# Autodesk Inventor assembly: Body
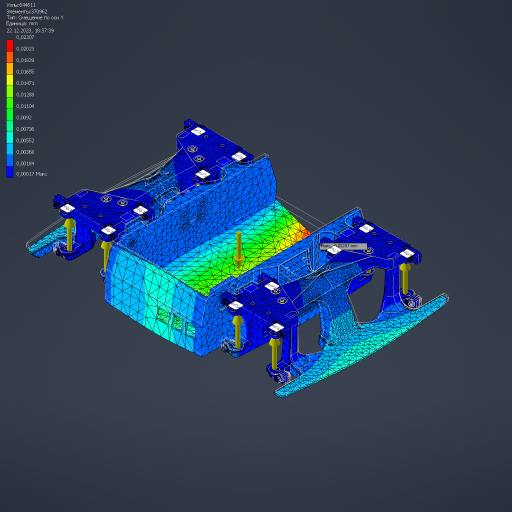
[picture p0: Inventor's stored thumbnail of the model, 512x512]
Saved by Autodesk Inventor 2023 (Build 270158000, 158)
## iProperties
Created: 2023-07-04
Part Number: Body
Document SubType Name: Assembly
Designer: khrip
Mass: 1155.31 g
Surface Area: 2834.72 cm^2
Volume: 832.799 cm^3
Density: 1.38726 g/cm^3
Author: khrip
## Documents named in this file (18)
- C:\GitHub\Botik\Body.iam
- C:\GitHub\Botik\BodyPlate.ipt
- C:\GitHub\Botik\BodyCupDiassembled.ipt
- C:\GitHub\Botik\BodyCupDiassembledMirrored.ipt
- C:\GitHub\Botik\Bumper.ipt
- C:\Users\khrip\OneDrive\Документы\Inventor\Content Center Files\R2023\ru-RU\GOST 11371-78  A\Шайба 3 ГОСТ 11371-78.ipt
- C:\Users\khrip\OneDrive\Документы\Inventor\Content Center Files\R2023\ru-RU\DIN 934\DIN 934 - M3 x 0,5.ipt
- C:\Users\khrip\OneDrive\Документы\Inventor\Content Center Files\R2023\ru-RU\DIN 912\DIN 912 - M3 x 0,5 x 10 x 8,75.ipt
- C:\GitHub\Botik\CrossBar.ipt
- C:\Users\khrip\OneDrive\Документы\Inventor\Content Center Files\R2023\ru-RU\GOST 17475-80 (2)\Винт 2.M4-6gx14 ГОСТ 17475-80.ipt
- C:\Users\khrip\OneDrive\Документы\Inventor\Content Center Files\R2023\ru-RU\GOST 11371-78  A\Шайба 4 ГОСТ 11371-78.ipt
- C:\Users\khrip\OneDrive\Документы\Inventor\Content Center Files\R2023\ru-RU\DIN 934\DIN 934 - M4 x 0,7.ipt
- C:\GitHub\Botik\Body\AIP\FEA\ek0i76urk.fins
- C:\GitHub\Botik\Body\AIP\FEA\ek0i76urk.fsat
- C:\GitHub\Botik\Body\AIP\FEA\ek0i76urk.ftes
- C:\GitHub\Botik\Body\AIP\FEA\ek0i76urk.fwiz
- C:\GitHub\Botik\Body\AIP\FEA\ek0i76v5s.fmsh
- C:\GitHub\Botik\Body\AIP\FEA\ek0i76v5t.fres
## Components (145 placed, 11 different names)
1. BodyPlate:1 — Совмещение:40, Заподлицо:14, Совмещение:41, Совмещение:42, Совмещение:43, Заподлицо:15, Совмещение:44, Заподлицо:16, Совмещение:45, Заподлицо:17, Совмещение:47, Совмещение:48, Вставка:4, Вставка:5, Вставка:9, Вставка:10, Вставка:12, Вставка:13, Вставка:15, Вставка:16, Вставка:17, Вставка:18, Вставка:19, Вставка:20, Вставка:24, Вставка:25, Вставка:27, Вставка:28
2. BodyCupDiassembled:1 — Совмещение:40, Заподлицо:14, Совмещение:41, Совмещение:51, Совмещение:52, Заподлицо:19, Вставка:30, Вставка:31, Вставка:32, Вставка:33, Вставка:34, Вставка:35, Совмещение:159, Совмещение:162, Совмещение:163, Совмещение:171, Совмещение:173
3. BodyCupDiassembled:2 — Совмещение:42, Совмещение:43, Заподлицо:15, Совмещение:49, Совмещение:50, Заподлицо:18, Совмещение:53, Совмещение:54, Совмещение:55, Совмещение:56, Вставка:21, Вставка:22, Вставка:23, Вставка:26, Совмещение:166, Совмещение:167, Совмещение:179, Совмещение:181
4. BodyCupDiassembledMirroredMirrored:1 — Заподлицо:17, Совмещение:47, Совмещение:48, Вставка:2, Вставка:3, Вставка:7, Вставка:8, Вставка:11, Вставка:14, Совмещение:168, Совмещение:169, Совмещение:183, Совмещение:185
5. BodyCupDiassembledMirroredMirrored:2 — Совмещение:44, Заподлицо:16, Совмещение:45, Вставка:39, Вставка:40, Вставка:42, Вставка:43, Вставка:44, Вставка:45, Совмещение:160, Совмещение:164, Совмещение:165, Совмещение:175, Совмещение:177
6. Bumper:1 — Совмещение:49, Совмещение:50, Заподлицо:18, Вставка:1, Вставка:6, Совмещение:57, Совмещение:58, Вставка:29, Совмещение:157, Совмещение:158
7. Bumper:2 — Совмещение:51, Совмещение:52, Заподлицо:19, Вставка:36, Вставка:37, Вставка:38, Вставка:41, Совмещение:161
8. CrossBar:1 — Вставка:54, Вставка:55, Вставка:56, Вставка:57, Вставка:58, Вставка:59, Вставка:60, Вставка:61, Совмещение:157, Совмещение:158
9. CrossBar:2 — Вставка:46, Вставка:47, Вставка:48, Вставка:49, Вставка:50, Вставка:51, Вставка:52, Вставка:53, Совмещение:159, Совмещение:160, Совмещение:161
10. DIN 934 - заменено на DIN EN 24032/28673/28674 M3:25 — Вставка:46
11. DIN 934 - заменено на DIN EN 24032/28673/28674 M3:26 — Вставка:47
12. DIN 934 - заменено на DIN EN 24032/28673/28674 M3:27 — Вставка:48
13. DIN 934 - заменено на DIN EN 24032/28673/28674 M3:28 — Вставка:49
14. DIN 934 - заменено на DIN EN 24032/28673/28674 M3:29 — Вставка:50
15. DIN 934 - заменено на DIN EN 24032/28673/28674 M3:30 — Вставка:51
16. DIN 934 - заменено на DIN EN 24032/28673/28674 M3:31 — Вставка:52
17. DIN 934 - заменено на DIN EN 24032/28673/28674 M3:32 — Вставка:53
18. DIN 934 - заменено на DIN EN 24032/28673/28674 M3:33 — Вставка:54
19. DIN 934 - заменено на DIN EN 24032/28673/28674 M3:34 — Вставка:55
20. DIN 934 - заменено на DIN EN 24032/28673/28674 M3:35 — Вставка:56
21. DIN 934 - заменено на DIN EN 24032/28673/28674 M3:36 — Вставка:57
22. DIN 934 - заменено на DIN EN 24032/28673/28674 M3:37 — Вставка:58
23. DIN 934 - заменено на DIN EN 24032/28673/28674 M3:38 — Вставка:59
24. DIN 934 - заменено на DIN EN 24032/28673/28674 M3:39 — Вставка:60
25. DIN 934 - заменено на DIN EN 24032/28673/28674 M3:40 — Вставка:61
26. Винт 2 ГОСТ 17475-80 M4 x 14:1 — Совмещение:162, Совмещение:170, Совмещение:196
27. Винт 2 ГОСТ 17475-80 M4 x 14:2 — Совмещение:163, Совмещение:172, Совмещение:194
28. Винт 2 ГОСТ 17475-80 M4 x 14:3 — Совмещение:164, Совмещение:176, Совмещение:200
29. Винт 2 ГОСТ 17475-80 M4 x 14:4 — Совмещение:165, Совмещение:174, Совмещение:198
30. Винт 2 ГОСТ 17475-80 M4 x 14:5 — Совмещение:166, Совмещение:178, Совмещение:192
31. Винт 2 ГОСТ 17475-80 M4 x 14:6 — Совмещение:167, Совмещение:180, Совмещение:190
32. Винт 2 ГОСТ 17475-80 M4 x 14:7 — Совмещение:168, Совмещение:182, Совмещение:186
33. Винт 2 ГОСТ 17475-80 M4 x 14:8 — Совмещение:169, Совмещение:184, Совмещение:188
34. Шайба  ГОСТ 11371-78 4,3:1 — Совмещение:170, Совмещение:171, Совмещение:197
35. Шайба  ГОСТ 11371-78 4,3:2 — Совмещение:172, Совмещение:173, Совмещение:195
36. Шайба  ГОСТ 11371-78 4,3:3 — Совмещение:174, Совмещение:175, Совмещение:199
37. Шайба  ГОСТ 11371-78 4,3:4 — Совмещение:176, Совмещение:177, Совмещение:201
38. Шайба  ГОСТ 11371-78 4,3:5 — Совмещение:178, Совмещение:179, Совмещение:193
39. Шайба  ГОСТ 11371-78 4,3:6 — Совмещение:180, Совмещение:181, Совмещение:191
40. Шайба  ГОСТ 11371-78 4,3:7 — Совмещение:182, Совмещение:183, Совмещение:187
41. Шайба  ГОСТ 11371-78 4,3:8 — Совмещение:184, Совмещение:185, Совмещение:189
42. DIN 934 - заменено на DIN EN 24032/28673/28674 M4:1 — Совмещение:186, Совмещение:187
43. DIN 934 - заменено на DIN EN 24032/28673/28674 M4:2 — Совмещение:188, Совмещение:189
44. DIN 934 - заменено на DIN EN 24032/28673/28674 M4:3 — Совмещение:190, Совмещение:191
45. DIN 934 - заменено на DIN EN 24032/28673/28674 M4:4 — Совмещение:192, Совмещение:193
46. DIN 934 - заменено на DIN EN 24032/28673/28674 M4:5 — Совмещение:194, Совмещение:195
47. DIN 934 - заменено на DIN EN 24032/28673/28674 M4:6 — Совмещение:196, Совмещение:197
48. DIN 934 - заменено на DIN EN 24032/28673/28674 M4:7 — Совмещение:198, Совмещение:199
49. DIN 934 - заменено на DIN EN 24032/28673/28674 M4:8 — Совмещение:200, Совмещение:201
50. Шайба  ГОСТ 11371-78 3,2:11 — Вставка:11, Совмещение:79, Совмещение:80
51. Шайба  ГОСТ 11371-78 3,2:12 — Вставка:12, Совмещение:81, Совмещение:82
52. Шайба  ГОСТ 11371-78 3,2:13 — Вставка:13, Совмещение:69, Совмещение:70
53. Шайба  ГОСТ 11371-78 3,2:14 — Вставка:14, Совмещение:124
54. Шайба  ГОСТ 11371-78 3,2:15 — Вставка:15, Совмещение:126
55. Шайба  ГОСТ 11371-78 3,2:16 — Вставка:16, Совмещение:118
56. Шайба  ГОСТ 11371-78 3,2:17 — Совмещение:53, Совмещение:54, Совмещение:71, Совмещение:72
57. Шайба  ГОСТ 11371-78 3,2:18 — Совмещение:55, Совмещение:56, Совмещение:73, Совмещение:74
58. Шайба  ГОСТ 11371-78 3,2:19 — Вставка:17, Совмещение:77, Совмещение:78
59. Шайба  ГОСТ 11371-78 3,2:20 — Вставка:18, Совмещение:63, Совмещение:64
60. Шайба  ГОСТ 11371-78 3,2:21 — Вставка:19, Совмещение:128
61. Шайба  ГОСТ 11371-78 3,2:22 — Вставка:20, Совмещение:112
62. Шайба  ГОСТ 11371-78 3,2:23 — Вставка:21, Совмещение:130
63. Шайба  ГОСТ 11371-78 3,2:24 — Вставка:22, Совмещение:96
64. Шайба  ГОСТ 11371-78 3,2:25 — Вставка:23, Совмещение:83, Совмещение:84
65. Шайба  ГОСТ 11371-78 3,2:26 — Вставка:24, Совмещение:85, Совмещение:86
66. Шайба  ГОСТ 11371-78 3,2:27 — Вставка:25, Совмещение:99, Совмещение:100
67. Шайба  ГОСТ 11371-78 3,2:28 — Вставка:26, Совмещение:142
68. Шайба  ГОСТ 11371-78 3,2:29 — Вставка:27, Совмещение:140
69. Шайба  ГОСТ 11371-78 3,2:30 — Вставка:28, Совмещение:152
70. Шайба  ГОСТ 11371-78 3,2:31 — Совмещение:57, Совмещение:58, Совмещение:75, Совмещение:76
71. Шайба  ГОСТ 11371-78 3,2:32 — Вставка:29, Совмещение:110
72. Шайба  ГОСТ 11371-78 3,2:33 — Вставка:30, Совмещение:101, Совмещение:102
73. Шайба  ГОСТ 11371-78 3,2:34 — Вставка:31, Совмещение:105, Совмещение:106
74. Шайба  ГОСТ 11371-78 3,2:35 — Вставка:32, Совмещение:136
75. Шайба  ГОСТ 11371-78 3,2:36 — Вставка:33, Совмещение:134
76. Шайба  ГОСТ 11371-78 3,2:37 — Вставка:34, Совмещение:67, Совмещение:68
77. Шайба  ГОСТ 11371-78 3,2:38 — Вставка:35, Совмещение:116
78. Шайба  ГОСТ 11371-78 3,2:39 — Вставка:36, Совмещение:132
79. Шайба  ГОСТ 11371-78 3,2:40 — Вставка:37, Совмещение:107, Совмещение:108
80. Шайба  ГОСТ 11371-78 3,2:41 — Вставка:38, Совмещение:65, Совмещение:66
81. Шайба  ГОСТ 11371-78 3,2:42 — Вставка:39, Совмещение:61, Совмещение:62
82. Шайба  ГОСТ 11371-78 3,2:43 — Вставка:40, Совмещение:59, Совмещение:60
83. Шайба  ГОСТ 11371-78 3,2:44 — Вставка:41, Совмещение:122
84. Шайба  ГОСТ 11371-78 3,2:45 — Вставка:42, Совмещение:120
85. Шайба  ГОСТ 11371-78 3,2:46 — Вставка:43, Совмещение:114
86. Шайба  ГОСТ 11371-78 3,2:47 — Вставка:44, Совмещение:138
87. Шайба  ГОСТ 11371-78 3,2:48 — Вставка:45, Совмещение:97, Совмещение:98
88. Шайба  ГОСТ 11371-78 3,2:1 — Вставка:1, Совмещение:89, Совмещение:90
89. Шайба  ГОСТ 11371-78 3,2:2 — Вставка:2, Совмещение:87, Совмещение:88
90. Шайба  ГОСТ 11371-78 3,2:3 — Вставка:3, Совмещение:91, Совмещение:92
91. Шайба  ГОСТ 11371-78 3,2:4 — Вставка:4, Совмещение:93, Совмещение:94
92. Шайба  ГОСТ 11371-78 3,2:5 — Вставка:5, Совмещение:103, Совмещение:104
93. Шайба  ГОСТ 11371-78 3,2:6 — Вставка:6, Совмещение:148
94. Шайба  ГОСТ 11371-78 3,2:7 — Вставка:7, Совмещение:150
95. Шайба  ГОСТ 11371-78 3,2:8 — Вставка:8, Совмещение:144
96. Шайба  ГОСТ 11371-78 3,2:9 — Вставка:9, Совмещение:146
97. Шайба  ГОСТ 11371-78 3,2:10 — Вставка:10, Совмещение:154
98. DIN 912 - заменено на DIN EN ISO 4762 M3 x 10:1 — Совмещение:59, Совмещение:60, Совмещение:113
99. DIN 912 - заменено на DIN EN ISO 4762 M3 x 10:2 — Совмещение:61, Совмещение:62, Совмещение:119
100. DIN 912 - заменено на DIN EN ISO 4762 M3 x 10:3 — Совмещение:63, Совмещение:64, Совмещение:111
101. DIN 912 - заменено на DIN EN ISO 4762 M3 x 10:4 — Совмещение:65, Совмещение:66, Совмещение:121
102. DIN 912 - заменено на DIN EN ISO 4762 M3 x 10:5 — Совмещение:67, Совмещение:68, Совмещение:115
103. DIN 912 - заменено на DIN EN ISO 4762 M3 x 10:6 — Совмещение:69, Совмещение:70, Совмещение:117
104. DIN 912 - заменено на DIN EN ISO 4762 M3 x 10:7 — Совмещение:71, Совмещение:72, Совмещение:129
105. DIN 912 - заменено на DIN EN ISO 4762 M3 x 10:8 — Совмещение:73, Совмещение:74, Совмещение:95
106. DIN 912 - заменено на DIN EN ISO 4762 M3 x 10:9 — Совмещение:75, Совмещение:76, Совмещение:109
107. DIN 912 - заменено на DIN EN ISO 4762 M3 x 10:10 — Совмещение:77, Совмещение:78, Совмещение:127
108. DIN 912 - заменено на DIN EN ISO 4762 M3 x 10:11 — Совмещение:79, Совмещение:80, Совмещение:123
109. DIN 912 - заменено на DIN EN ISO 4762 M3 x 10:12 — Совмещение:81, Совмещение:82, Совмещение:125
110. DIN 912 - заменено на DIN EN ISO 4762 M3 x 10:13 — Совмещение:83, Совмещение:84, Совмещение:141
111. DIN 912 - заменено на DIN EN ISO 4762 M3 x 10:14 — Совмещение:85, Совмещение:86, Совмещение:139
112. DIN 912 - заменено на DIN EN ISO 4762 M3 x 10:15 — Совмещение:87, Совмещение:88, Совмещение:149
113. DIN 912 - заменено на DIN EN ISO 4762 M3 x 10:16 — Совмещение:89, Совмещение:90, Совмещение:147
114. DIN 912 - заменено на DIN EN ISO 4762 M3 x 10:17 — Совмещение:91, Совмещение:92, Совмещение:143
115. DIN 912 - заменено на DIN EN ISO 4762 M3 x 10:18 — Совмещение:93, Совмещение:94, Совмещение:145
116. DIN 912 - заменено на DIN EN ISO 4762 M3 x 10:19 — Совмещение:97, Совмещение:98, Совмещение:137
117. DIN 912 - заменено на DIN EN ISO 4762 M3 x 10:20 — Совмещение:99, Совмещение:100, Совмещение:151
118. DIN 912 - заменено на DIN EN ISO 4762 M3 x 10:21 — Совмещение:101, Совмещение:102, Совмещение:135
119. DIN 912 - заменено на DIN EN ISO 4762 M3 x 10:22 — Совмещение:103, Совмещение:104, Совмещение:153
120. DIN 912 - заменено на DIN EN ISO 4762 M3 x 10:23 — Совмещение:105, Совмещение:106, Совмещение:133
121. DIN 912 - заменено на DIN EN ISO 4762 M3 x 10:24 — Совмещение:107, Совмещение:108, Совмещение:131
122. DIN 934 - заменено на DIN EN 24032/28673/28674 M3:2 — Совмещение:109, Совмещение:110
123. DIN 934 - заменено на DIN EN 24032/28673/28674 M3:3 — Совмещение:111, Совмещение:112
124. DIN 934 - заменено на DIN EN 24032/28673/28674 M3:4 — Совмещение:113, Совмещение:114
125. DIN 934 - заменено на DIN EN 24032/28673/28674 M3:5 — Совмещение:115, Совмещение:116
126. DIN 934 - заменено на DIN EN 24032/28673/28674 M3:6 — Совмещение:117, Совмещение:118
127. DIN 934 - заменено на DIN EN 24032/28673/28674 M3:7 — Совмещение:119, Совмещение:120
128. DIN 934 - заменено на DIN EN 24032/28673/28674 M3:8 — Совмещение:121, Совмещение:122
129. DIN 934 - заменено на DIN EN 24032/28673/28674 M3:9 — Совмещение:123, Совмещение:124
130. DIN 934 - заменено на DIN EN 24032/28673/28674 M3:10 — Совмещение:125, Совмещение:126
131. DIN 934 - заменено на DIN EN 24032/28673/28674 M3:11 — Совмещение:127, Совмещение:128
132. DIN 934 - заменено на DIN EN 24032/28673/28674 M3:12 — Совмещение:129, Совмещение:130
133. DIN 934 - заменено на DIN EN 24032/28673/28674 M3:13 — Совмещение:131, Совмещение:132
134. DIN 934 - заменено на DIN EN 24032/28673/28674 M3:14 — Совмещение:133, Совмещение:134
135. DIN 934 - заменено на DIN EN 24032/28673/28674 M3:15 — Совмещение:135, Совмещение:136
136. DIN 934 - заменено на DIN EN 24032/28673/28674 M3:16 — Совмещение:137, Совмещение:138
137. DIN 934 - заменено на DIN EN 24032/28673/28674 M3:17 — Совмещение:139, Совмещение:140
138. DIN 934 - заменено на DIN EN 24032/28673/28674 M3:18 — Совмещение:141, Совмещение:142
139. DIN 934 - заменено на DIN EN 24032/28673/28674 M3:19 — Совмещение:143, Совмещение:144
140. DIN 934 - заменено на DIN EN 24032/28673/28674 M3:20 — Совмещение:145, Совмещение:146
141. DIN 934 - заменено на DIN EN 24032/28673/28674 M3:21 — Совмещение:147, Совмещение:148
142. DIN 934 - заменено на DIN EN 24032/28673/28674 M3:22 — Совмещение:149, Совмещение:150
143. DIN 934 - заменено на DIN EN 24032/28673/28674 M3:23 — Совмещение:151, Совмещение:152
144. DIN 934 - заменено на DIN EN 24032/28673/28674 M3:24 — Совмещение:153, Совмещение:154
145. DIN 934 - заменено на DIN EN 24032/28673/28674 M3:1 — Совмещение:95, Совмещение:96
## Relationships (226: Mate 159, Insert 61, Flush 6)
- Совмещение:40 [Mate]: BodyPlate:1 ↔ BodyCupDiassembled:1
- Заподлицо:14 [Flush]: BodyPlate:1 ↔ BodyCupDiassembled:1
- Совмещение:41 [Mate]: BodyPlate:1 ↔ BodyCupDiassembled:1
- Совмещение:42 [Mate]: BodyPlate:1 ↔ BodyCupDiassembled:2
- Совмещение:43 [Mate]: BodyPlate:1 ↔ BodyCupDiassembled:2
- Заподлицо:15 [Flush]: BodyPlate:1 ↔ BodyCupDiassembled:2
- Совмещение:44 [Mate]: BodyPlate:1 ↔ BodyCupDiassembledMirroredMirrored:2
- Заподлицо:16 [Flush]: BodyPlate:1 ↔ BodyCupDiassembledMirroredMirrored:2
- Совмещение:45 [Mate]: BodyPlate:1 ↔ BodyCupDiassembledMirroredMirrored:2
- Заподлицо:17 [Flush]: BodyPlate:1 ↔ BodyCupDiassembledMirroredMirrored:1
- Совмещение:47 [Mate]: BodyPlate:1 ↔ BodyCupDiassembledMirroredMirrored:1
- Совмещение:48 [Mate]: BodyPlate:1 ↔ BodyCupDiassembledMirroredMirrored:1
- Совмещение:49 [Mate]: BodyCupDiassembled:2 ↔ Bumper:1
- Совмещение:50 [Mate]: BodyCupDiassembled:2 ↔ Bumper:1
- Заподлицо:18 [Flush]: BodyCupDiassembled:2 ↔ Bumper:1
- Совмещение:51 [Mate]: BodyCupDiassembled:1 ↔ Bumper:2
- Совмещение:52 [Mate]: BodyCupDiassembled:1 ↔ Bumper:2
- Заподлицо:19 [Flush]: BodyCupDiassembled:1 ↔ Bumper:2
- Вставка:1 [Insert]: Bumper:1 ↔ Шайба  ГОСТ 11371-78 3,2:1
- Вставка:2 [Insert]: BodyCupDiassembledMirroredMirrored:1 ↔ Шайба  ГОСТ 11371-78 3,2:2
- Вставка:3 [Insert]: BodyCupDiassembledMirroredMirrored:1 ↔ Шайба  ГОСТ 11371-78 3,2:3
- Вставка:4 [Insert]: BodyPlate:1 ↔ Шайба  ГОСТ 11371-78 3,2:4
- Вставка:5 [Insert]: BodyPlate:1 ↔ Шайба  ГОСТ 11371-78 3,2:5
- Вставка:6 [Insert]: Bumper:1 ↔ Шайба  ГОСТ 11371-78 3,2:6
- Вставка:7 [Insert]: BodyCupDiassembledMirroredMirrored:1 ↔ Шайба  ГОСТ 11371-78 3,2:7
- Вставка:8 [Insert]: BodyCupDiassembledMirroredMirrored:1 ↔ Шайба  ГОСТ 11371-78 3,2:8
- Вставка:9 [Insert]: BodyPlate:1 ↔ Шайба  ГОСТ 11371-78 3,2:9
- Вставка:10 [Insert]: BodyPlate:1 ↔ Шайба  ГОСТ 11371-78 3,2:10
- Вставка:11 [Insert]: BodyCupDiassembledMirroredMirrored:1 ↔ Шайба  ГОСТ 11371-78 3,2:11
- Вставка:12 [Insert]: BodyPlate:1 ↔ Шайба  ГОСТ 11371-78 3,2:12
- Вставка:13 [Insert]: BodyPlate:1 ↔ Шайба  ГОСТ 11371-78 3,2:13
- Вставка:14 [Insert]: BodyCupDiassembledMirroredMirrored:1 ↔ Шайба  ГОСТ 11371-78 3,2:14
- Вставка:15 [Insert]: BodyPlate:1 ↔ Шайба  ГОСТ 11371-78 3,2:15
- Вставка:16 [Insert]: BodyPlate:1 ↔ Шайба  ГОСТ 11371-78 3,2:16
- Совмещение:53 [Mate]: BodyCupDiassembled:2 ↔ Шайба  ГОСТ 11371-78 3,2:17
- Совмещение:54 [Mate]: BodyCupDiassembled:2 ↔ Шайба  ГОСТ 11371-78 3,2:17
- Совмещение:55 [Mate]: BodyCupDiassembled:2 ↔ Шайба  ГОСТ 11371-78 3,2:18
- Совмещение:56 [Mate]: BodyCupDiassembled:2 ↔ Шайба  ГОСТ 11371-78 3,2:18
- Вставка:17 [Insert]: BodyPlate:1 ↔ Шайба  ГОСТ 11371-78 3,2:19
- Вставка:18 [Insert]: BodyPlate:1 ↔ Шайба  ГОСТ 11371-78 3,2:20
- Вставка:19 [Insert]: BodyPlate:1 ↔ Шайба  ГОСТ 11371-78 3,2:21
- Вставка:20 [Insert]: BodyPlate:1 ↔ Шайба  ГОСТ 11371-78 3,2:22
- Вставка:21 [Insert]: BodyCupDiassembled:2 ↔ Шайба  ГОСТ 11371-78 3,2:23
- Вставка:22 [Insert]: BodyCupDiassembled:2 ↔ Шайба  ГОСТ 11371-78 3,2:24
- Вставка:23 [Insert]: BodyCupDiassembled:2 ↔ Шайба  ГОСТ 11371-78 3,2:25
- Вставка:24 [Insert]: BodyPlate:1 ↔ Шайба  ГОСТ 11371-78 3,2:26
- Вставка:25 [Insert]: BodyPlate:1 ↔ Шайба  ГОСТ 11371-78 3,2:27
- Вставка:26 [Insert]: BodyCupDiassembled:2 ↔ Шайба  ГОСТ 11371-78 3,2:28
- Вставка:27 [Insert]: BodyPlate:1 ↔ Шайба  ГОСТ 11371-78 3,2:29
- Вставка:28 [Insert]: BodyPlate:1 ↔ Шайба  ГОСТ 11371-78 3,2:30
- Совмещение:57 [Mate]: Bumper:1 ↔ Шайба  ГОСТ 11371-78 3,2:31
- Совмещение:58 [Mate]: Bumper:1 ↔ Шайба  ГОСТ 11371-78 3,2:31
- Вставка:29 [Insert]: Bumper:1 ↔ Шайба  ГОСТ 11371-78 3,2:32
- Вставка:30 [Insert]: BodyCupDiassembled:1 ↔ Шайба  ГОСТ 11371-78 3,2:33
- Вставка:31 [Insert]: BodyCupDiassembled:1 ↔ Шайба  ГОСТ 11371-78 3,2:34
- Вставка:32 [Insert]: BodyCupDiassembled:1 ↔ Шайба  ГОСТ 11371-78 3,2:35
- Вставка:33 [Insert]: BodyCupDiassembled:1 ↔ Шайба  ГОСТ 11371-78 3,2:36
- Вставка:34 [Insert]: BodyCupDiassembled:1 ↔ Шайба  ГОСТ 11371-78 3,2:37
- Вставка:35 [Insert]: BodyCupDiassembled:1 ↔ Шайба  ГОСТ 11371-78 3,2:38
- Вставка:36 [Insert]: Bumper:2 ↔ Шайба  ГОСТ 11371-78 3,2:39
- Вставка:37 [Insert]: Bumper:2 ↔ Шайба  ГОСТ 11371-78 3,2:40
- Вставка:38 [Insert]: Bumper:2 ↔ Шайба  ГОСТ 11371-78 3,2:41
- Вставка:39 [Insert]: BodyCupDiassembledMirroredMirrored:2 ↔ Шайба  ГОСТ 11371-78 3,2:42
- Вставка:40 [Insert]: BodyCupDiassembledMirroredMirrored:2 ↔ Шайба  ГОСТ 11371-78 3,2:43
- Вставка:41 [Insert]: Bumper:2 ↔ Шайба  ГОСТ 11371-78 3,2:44
- Вставка:42 [Insert]: BodyCupDiassembledMirroredMirrored:2 ↔ Шайба  ГОСТ 11371-78 3,2:45
- Вставка:43 [Insert]: BodyCupDiassembledMirroredMirrored:2 ↔ Шайба  ГОСТ 11371-78 3,2:46
- Вставка:44 [Insert]: BodyCupDiassembledMirroredMirrored:2 ↔ Шайба  ГОСТ 11371-78 3,2:47
- Вставка:45 [Insert]: BodyCupDiassembledMirroredMirrored:2 ↔ Шайба  ГОСТ 11371-78 3,2:48
- Совмещение:59 [Mate]: Шайба  ГОСТ 11371-78 3,2:43 ↔ DIN 912 - заменено на DIN EN ISO 4762 M3 x 10:1
- Совмещение:60 [Mate]: Шайба  ГОСТ 11371-78 3,2:43 ↔ DIN 912 - заменено на DIN EN ISO 4762 M3 x 10:1
- Совмещение:61 [Mate]: Шайба  ГОСТ 11371-78 3,2:42 ↔ DIN 912 - заменено на DIN EN ISO 4762 M3 x 10:2
- Совмещение:62 [Mate]: Шайба  ГОСТ 11371-78 3,2:42 ↔ DIN 912 - заменено на DIN EN ISO 4762 M3 x 10:2
- Совмещение:63 [Mate]: Шайба  ГОСТ 11371-78 3,2:20 ↔ DIN 912 - заменено на DIN EN ISO 4762 M3 x 10:3
- Совмещение:64 [Mate]: Шайба  ГОСТ 11371-78 3,2:20 ↔ DIN 912 - заменено на DIN EN ISO 4762 M3 x 10:3
- Совмещение:65 [Mate]: Шайба  ГОСТ 11371-78 3,2:41 ↔ DIN 912 - заменено на DIN EN ISO 4762 M3 x 10:4
- Совмещение:66 [Mate]: Шайба  ГОСТ 11371-78 3,2:41 ↔ DIN 912 - заменено на DIN EN ISO 4762 M3 x 10:4
- Совмещение:67 [Mate]: Шайба  ГОСТ 11371-78 3,2:37 ↔ DIN 912 - заменено на DIN EN ISO 4762 M3 x 10:5
- Совмещение:68 [Mate]: Шайба  ГОСТ 11371-78 3,2:37 ↔ DIN 912 - заменено на DIN EN ISO 4762 M3 x 10:5
- Совмещение:69 [Mate]: Шайба  ГОСТ 11371-78 3,2:13 ↔ DIN 912 - заменено на DIN EN ISO 4762 M3 x 10:6
- Совмещение:70 [Mate]: Шайба  ГОСТ 11371-78 3,2:13 ↔ DIN 912 - заменено на DIN EN ISO 4762 M3 x 10:6
- Совмещение:71 [Mate]: Шайба  ГОСТ 11371-78 3,2:17 ↔ DIN 912 - заменено на DIN EN ISO 4762 M3 x 10:7
- Совмещение:72 [Mate]: Шайба  ГОСТ 11371-78 3,2:17 ↔ DIN 912 - заменено на DIN EN ISO 4762 M3 x 10:7
- Совмещение:73 [Mate]: Шайба  ГОСТ 11371-78 3,2:18 ↔ DIN 912 - заменено на DIN EN ISO 4762 M3 x 10:8
- Совмещение:74 [Mate]: Шайба  ГОСТ 11371-78 3,2:18 ↔ DIN 912 - заменено на DIN EN ISO 4762 M3 x 10:8
- Совмещение:75 [Mate]: Шайба  ГОСТ 11371-78 3,2:31 ↔ DIN 912 - заменено на DIN EN ISO 4762 M3 x 10:9
- Совмещение:76 [Mate]: Шайба  ГОСТ 11371-78 3,2:31 ↔ DIN 912 - заменено на DIN EN ISO 4762 M3 x 10:9
- Совмещение:77 [Mate]: Шайба  ГОСТ 11371-78 3,2:19 ↔ DIN 912 - заменено на DIN EN ISO 4762 M3 x 10:10
- Совмещение:78 [Mate]: Шайба  ГОСТ 11371-78 3,2:19 ↔ DIN 912 - заменено на DIN EN ISO 4762 M3 x 10:10
- Совмещение:79 [Mate]: Шайба  ГОСТ 11371-78 3,2:11 ↔ DIN 912 - заменено на DIN EN ISO 4762 M3 x 10:11
- Совмещение:80 [Mate]: Шайба  ГОСТ 11371-78 3,2:11 ↔ DIN 912 - заменено на DIN EN ISO 4762 M3 x 10:11
- Совмещение:81 [Mate]: Шайба  ГОСТ 11371-78 3,2:12 ↔ DIN 912 - заменено на DIN EN ISO 4762 M3 x 10:12
- Совмещение:82 [Mate]: Шайба  ГОСТ 11371-78 3,2:12 ↔ DIN 912 - заменено на DIN EN ISO 4762 M3 x 10:12
- Совмещение:83 [Mate]: Шайба  ГОСТ 11371-78 3,2:25 ↔ DIN 912 - заменено на DIN EN ISO 4762 M3 x 10:13
- Совмещение:84 [Mate]: Шайба  ГОСТ 11371-78 3,2:25 ↔ DIN 912 - заменено на DIN EN ISO 4762 M3 x 10:13
- Совмещение:85 [Mate]: Шайба  ГОСТ 11371-78 3,2:26 ↔ DIN 912 - заменено на DIN EN ISO 4762 M3 x 10:14
- Совмещение:86 [Mate]: Шайба  ГОСТ 11371-78 3,2:26 ↔ DIN 912 - заменено на DIN EN ISO 4762 M3 x 10:14
- Совмещение:87 [Mate]: Шайба  ГОСТ 11371-78 3,2:2 ↔ DIN 912 - заменено на DIN EN ISO 4762 M3 x 10:15
- Совмещение:88 [Mate]: Шайба  ГОСТ 11371-78 3,2:2 ↔ DIN 912 - заменено на DIN EN ISO 4762 M3 x 10:15
- Совмещение:89 [Mate]: Шайба  ГОСТ 11371-78 3,2:1 ↔ DIN 912 - заменено на DIN EN ISO 4762 M3 x 10:16
- Совмещение:90 [Mate]: Шайба  ГОСТ 11371-78 3,2:1 ↔ DIN 912 - заменено на DIN EN ISO 4762 M3 x 10:16
- Совмещение:91 [Mate]: Шайба  ГОСТ 11371-78 3,2:3 ↔ DIN 912 - заменено на DIN EN ISO 4762 M3 x 10:17
- Совмещение:92 [Mate]: Шайба  ГОСТ 11371-78 3,2:3 ↔ DIN 912 - заменено на DIN EN ISO 4762 M3 x 10:17
- Совмещение:93 [Mate]: Шайба  ГОСТ 11371-78 3,2:4 ↔ DIN 912 - заменено на DIN EN ISO 4762 M3 x 10:18
- Совмещение:94 [Mate]: Шайба  ГОСТ 11371-78 3,2:4 ↔ DIN 912 - заменено на DIN EN ISO 4762 M3 x 10:18
- Совмещение:95 [Mate]: DIN 912 - заменено на DIN EN ISO 4762 M3 x 10:8 ↔ DIN 934 - заменено на DIN EN 24032/28673/28674 M3:1
- Совмещение:96 [Mate]: Шайба  ГОСТ 11371-78 3,2:24 ↔ DIN 934 - заменено на DIN EN 24032/28673/28674 M3:1
- Совмещение:97 [Mate]: Шайба  ГОСТ 11371-78 3,2:48 ↔ DIN 912 - заменено на DIN EN ISO 4762 M3 x 10:19
- Совмещение:98 [Mate]: Шайба  ГОСТ 11371-78 3,2:48 ↔ DIN 912 - заменено на DIN EN ISO 4762 M3 x 10:19
- Совмещение:99 [Mate]: Шайба  ГОСТ 11371-78 3,2:27 ↔ DIN 912 - заменено на DIN EN ISO 4762 M3 x 10:20
- Совмещение:100 [Mate]: Шайба  ГОСТ 11371-78 3,2:27 ↔ DIN 912 - заменено на DIN EN ISO 4762 M3 x 10:20
- Совмещение:101 [Mate]: Шайба  ГОСТ 11371-78 3,2:33 ↔ DIN 912 - заменено на DIN EN ISO 4762 M3 x 10:21
- Совмещение:102 [Mate]: Шайба  ГОСТ 11371-78 3,2:33 ↔ DIN 912 - заменено на DIN EN ISO 4762 M3 x 10:21
- Совмещение:103 [Mate]: Шайба  ГОСТ 11371-78 3,2:5 ↔ DIN 912 - заменено на DIN EN ISO 4762 M3 x 10:22
- Совмещение:104 [Mate]: Шайба  ГОСТ 11371-78 3,2:5 ↔ DIN 912 - заменено на DIN EN ISO 4762 M3 x 10:22
- Совмещение:105 [Mate]: Шайба  ГОСТ 11371-78 3,2:34 ↔ DIN 912 - заменено на DIN EN ISO 4762 M3 x 10:23
- Совмещение:106 [Mate]: Шайба  ГОСТ 11371-78 3,2:34 ↔ DIN 912 - заменено на DIN EN ISO 4762 M3 x 10:23
- Совмещение:107 [Mate]: Шайба  ГОСТ 11371-78 3,2:40 ↔ DIN 912 - заменено на DIN EN ISO 4762 M3 x 10:24
- Совмещение:108 [Mate]: Шайба  ГОСТ 11371-78 3,2:40 ↔ DIN 912 - заменено на DIN EN ISO 4762 M3 x 10:24
- Совмещение:109 [Mate]: DIN 912 - заменено на DIN EN ISO 4762 M3 x 10:9 ↔ DIN 934 - заменено на DIN EN 24032/28673/28674 M3:2
- Совмещение:110 [Mate]: Шайба  ГОСТ 11371-78 3,2:32 ↔ DIN 934 - заменено на DIN EN 24032/28673/28674 M3:2
- Совмещение:111 [Mate]: DIN 912 - заменено на DIN EN ISO 4762 M3 x 10:3 ↔ DIN 934 - заменено на DIN EN 24032/28673/28674 M3:3
- Совмещение:112 [Mate]: Шайба  ГОСТ 11371-78 3,2:22 ↔ DIN 934 - заменено на DIN EN 24032/28673/28674 M3:3
- Совмещение:113 [Mate]: DIN 912 - заменено на DIN EN ISO 4762 M3 x 10:1 ↔ DIN 934 - заменено на DIN EN 24032/28673/28674 M3:4
- Совмещение:114 [Mate]: Шайба  ГОСТ 11371-78 3,2:46 ↔ DIN 934 - заменено на DIN EN 24032/28673/28674 M3:4
- Совмещение:115 [Mate]: DIN 912 - заменено на DIN EN ISO 4762 M3 x 10:5 ↔ DIN 934 - заменено на DIN EN 24032/28673/28674 M3:5
- Совмещение:116 [Mate]: Шайба  ГОСТ 11371-78 3,2:38 ↔ DIN 934 - заменено на DIN EN 24032/28673/28674 M3:5
- Совмещение:117 [Mate]: DIN 912 - заменено на DIN EN ISO 4762 M3 x 10:6 ↔ DIN 934 - заменено на DIN EN 24032/28673/28674 M3:6
- Совмещение:118 [Mate]: Шайба  ГОСТ 11371-78 3,2:16 ↔ DIN 934 - заменено на DIN EN 24032/28673/28674 M3:6
- Совмещение:119 [Mate]: DIN 912 - заменено на DIN EN ISO 4762 M3 x 10:2 ↔ DIN 934 - заменено на DIN EN 24032/28673/28674 M3:7
- Совмещение:120 [Mate]: Шайба  ГОСТ 11371-78 3,2:45 ↔ DIN 934 - заменено на DIN EN 24032/28673/28674 M3:7
- Совмещение:121 [Mate]: DIN 912 - заменено на DIN EN ISO 4762 M3 x 10:4 ↔ DIN 934 - заменено на DIN EN 24032/28673/28674 M3:8
- Совмещение:122 [Mate]: Шайба  ГОСТ 11371-78 3,2:44 ↔ DIN 934 - заменено на DIN EN 24032/28673/28674 M3:8
- Совмещение:123 [Mate]: DIN 912 - заменено на DIN EN ISO 4762 M3 x 10:11 ↔ DIN 934 - заменено на DIN EN 24032/28673/28674 M3:9
- Совмещение:124 [Mate]: Шайба  ГОСТ 11371-78 3,2:14 ↔ DIN 934 - заменено на DIN EN 24032/28673/28674 M3:9
- Совмещение:125 [Mate]: DIN 912 - заменено на DIN EN ISO 4762 M3 x 10:12 ↔ DIN 934 - заменено на DIN EN 24032/28673/28674 M3:10
- Совмещение:126 [Mate]: Шайба  ГОСТ 11371-78 3,2:15 ↔ DIN 934 - заменено на DIN EN 24032/28673/28674 M3:10
- Совмещение:127 [Mate]: DIN 912 - заменено на DIN EN ISO 4762 M3 x 10:10 ↔ DIN 934 - заменено на DIN EN 24032/28673/28674 M3:11
- Совмещение:128 [Mate]: Шайба  ГОСТ 11371-78 3,2:21 ↔ DIN 934 - заменено на DIN EN 24032/28673/28674 M3:11
- Совмещение:129 [Mate]: DIN 912 - заменено на DIN EN ISO 4762 M3 x 10:7 ↔ DIN 934 - заменено на DIN EN 24032/28673/28674 M3:12
- Совмещение:130 [Mate]: Шайба  ГОСТ 11371-78 3,2:23 ↔ DIN 934 - заменено на DIN EN 24032/28673/28674 M3:12
- Совмещение:131 [Mate]: DIN 912 - заменено на DIN EN ISO 4762 M3 x 10:24 ↔ DIN 934 - заменено на DIN EN 24032/28673/28674 M3:13
- Совмещение:132 [Mate]: Шайба  ГОСТ 11371-78 3,2:39 ↔ DIN 934 - заменено на DIN EN 24032/28673/28674 M3:13
- Совмещение:133 [Mate]: DIN 912 - заменено на DIN EN ISO 4762 M3 x 10:23 ↔ DIN 934 - заменено на DIN EN 24032/28673/28674 M3:14
- Совмещение:134 [Mate]: Шайба  ГОСТ 11371-78 3,2:36 ↔ DIN 934 - заменено на DIN EN 24032/28673/28674 M3:14
- Совмещение:135 [Mate]: DIN 912 - заменено на DIN EN ISO 4762 M3 x 10:21 ↔ DIN 934 - заменено на DIN EN 24032/28673/28674 M3:15
- Совмещение:136 [Mate]: Шайба  ГОСТ 11371-78 3,2:35 ↔ DIN 934 - заменено на DIN EN 24032/28673/28674 M3:15
- Совмещение:137 [Mate]: DIN 912 - заменено на DIN EN ISO 4762 M3 x 10:19 ↔ DIN 934 - заменено на DIN EN 24032/28673/28674 M3:16
- Совмещение:138 [Mate]: Шайба  ГОСТ 11371-78 3,2:47 ↔ DIN 934 - заменено на DIN EN 24032/28673/28674 M3:16
- Совмещение:139 [Mate]: DIN 912 - заменено на DIN EN ISO 4762 M3 x 10:14 ↔ DIN 934 - заменено на DIN EN 24032/28673/28674 M3:17
- Совмещение:140 [Mate]: Шайба  ГОСТ 11371-78 3,2:29 ↔ DIN 934 - заменено на DIN EN 24032/28673/28674 M3:17
- Совмещение:141 [Mate]: DIN 912 - заменено на DIN EN ISO 4762 M3 x 10:13 ↔ DIN 934 - заменено на DIN EN 24032/28673/28674 M3:18
- Совмещение:142 [Mate]: Шайба  ГОСТ 11371-78 3,2:28 ↔ DIN 934 - заменено на DIN EN 24032/28673/28674 M3:18
- Совмещение:143 [Mate]: DIN 912 - заменено на DIN EN ISO 4762 M3 x 10:17 ↔ DIN 934 - заменено на DIN EN 24032/28673/28674 M3:19
- Совмещение:144 [Mate]: Шайба  ГОСТ 11371-78 3,2:8 ↔ DIN 934 - заменено на DIN EN 24032/28673/28674 M3:19
- Совмещение:145 [Mate]: DIN 912 - заменено на DIN EN ISO 4762 M3 x 10:18 ↔ DIN 934 - заменено на DIN EN 24032/28673/28674 M3:20
- Совмещение:146 [Mate]: Шайба  ГОСТ 11371-78 3,2:9 ↔ DIN 934 - заменено на DIN EN 24032/28673/28674 M3:20
- Совмещение:147 [Mate]: DIN 912 - заменено на DIN EN ISO 4762 M3 x 10:16 ↔ DIN 934 - заменено на DIN EN 24032/28673/28674 M3:21
- Совмещение:148 [Mate]: Шайба  ГОСТ 11371-78 3,2:6 ↔ DIN 934 - заменено на DIN EN 24032/28673/28674 M3:21
- Совмещение:149 [Mate]: DIN 912 - заменено на DIN EN ISO 4762 M3 x 10:15 ↔ DIN 934 - заменено на DIN EN 24032/28673/28674 M3:22
- Совмещение:150 [Mate]: Шайба  ГОСТ 11371-78 3,2:7 ↔ DIN 934 - заменено на DIN EN 24032/28673/28674 M3:22
- Совмещение:151 [Mate]: DIN 912 - заменено на DIN EN ISO 4762 M3 x 10:20 ↔ DIN 934 - заменено на DIN EN 24032/28673/28674 M3:23
- Совмещение:152 [Mate]: Шайба  ГОСТ 11371-78 3,2:30 ↔ DIN 934 - заменено на DIN EN 24032/28673/28674 M3:23
- Совмещение:153 [Mate]: DIN 912 - заменено на DIN EN ISO 4762 M3 x 10:22 ↔ DIN 934 - заменено на DIN EN 24032/28673/28674 M3:24
- Совмещение:154 [Mate]: Шайба  ГОСТ 11371-78 3,2:10 ↔ DIN 934 - заменено на DIN EN 24032/28673/28674 M3:24
- Вставка:46 [Insert]: CrossBar:2 ↔ DIN 934 - заменено на DIN EN 24032/28673/28674 M3:25
- Вставка:47 [Insert]: CrossBar:2 ↔ DIN 934 - заменено на DIN EN 24032/28673/28674 M3:26
- Вставка:48 [Insert]: CrossBar:2 ↔ DIN 934 - заменено на DIN EN 24032/28673/28674 M3:27
- Вставка:49 [Insert]: CrossBar:2 ↔ DIN 934 - заменено на DIN EN 24032/28673/28674 M3:28
- Вставка:50 [Insert]: CrossBar:2 ↔ DIN 934 - заменено на DIN EN 24032/28673/28674 M3:29
- Вставка:51 [Insert]: CrossBar:2 ↔ DIN 934 - заменено на DIN EN 24032/28673/28674 M3:30
- Вставка:52 [Insert]: CrossBar:2 ↔ DIN 934 - заменено на DIN EN 24032/28673/28674 M3:31
- Вставка:53 [Insert]: CrossBar:2 ↔ DIN 934 - заменено на DIN EN 24032/28673/28674 M3:32
- Вставка:54 [Insert]: CrossBar:1 ↔ DIN 934 - заменено на DIN EN 24032/28673/28674 M3:33
- Вставка:55 [Insert]: CrossBar:1 ↔ DIN 934 - заменено на DIN EN 24032/28673/28674 M3:34
- Вставка:56 [Insert]: CrossBar:1 ↔ DIN 934 - заменено на DIN EN 24032/28673/28674 M3:35
- Вставка:57 [Insert]: CrossBar:1 ↔ DIN 934 - заменено на DIN EN 24032/28673/28674 M3:36
- Вставка:58 [Insert]: CrossBar:1 ↔ DIN 934 - заменено на DIN EN 24032/28673/28674 M3:37
- Вставка:59 [Insert]: CrossBar:1 ↔ DIN 934 - заменено на DIN EN 24032/28673/28674 M3:38
- Вставка:60 [Insert]: CrossBar:1 ↔ DIN 934 - заменено на DIN EN 24032/28673/28674 M3:39
- Вставка:61 [Insert]: CrossBar:1 ↔ DIN 934 - заменено на DIN EN 24032/28673/28674 M3:40
- Совмещение:157 [Mate]: Bumper:1 ↔ CrossBar:1
- Совмещение:158 [Mate]: Bumper:1 ↔ CrossBar:1
- Совмещение:159 [Mate]: BodyCupDiassembled:1 ↔ CrossBar:2
- Совмещение:160 [Mate]: BodyCupDiassembledMirroredMirrored:2 ↔ CrossBar:2
- Совмещение:161 [Mate]: Bumper:2 ↔ CrossBar:2
- Совмещение:162 [Mate]: BodyCupDiassembled:1 ↔ Винт 2 ГОСТ 17475-80 M4 x 14:1
- Совмещение:163 [Mate]: BodyCupDiassembled:1 ↔ Винт 2 ГОСТ 17475-80 M4 x 14:2
- Совмещение:164 [Mate]: BodyCupDiassembledMirroredMirrored:2 ↔ Винт 2 ГОСТ 17475-80 M4 x 14:3
- Совмещение:165 [Mate]: BodyCupDiassembledMirroredMirrored:2 ↔ Винт 2 ГОСТ 17475-80 M4 x 14:4
- Совмещение:166 [Mate]: BodyCupDiassembled:2 ↔ Винт 2 ГОСТ 17475-80 M4 x 14:5
- Совмещение:167 [Mate]: BodyCupDiassembled:2 ↔ Винт 2 ГОСТ 17475-80 M4 x 14:6
- Совмещение:168 [Mate]: BodyCupDiassembledMirroredMirrored:1 ↔ Винт 2 ГОСТ 17475-80 M4 x 14:7
- Совмещение:169 [Mate]: BodyCupDiassembledMirroredMirrored:1 ↔ Винт 2 ГОСТ 17475-80 M4 x 14:8
- Совмещение:170 [Mate]: Винт 2 ГОСТ 17475-80 M4 x 14:1 ↔ Шайба  ГОСТ 11371-78 4,3:1
- Совмещение:171 [Mate]: BodyCupDiassembled:1 ↔ Шайба  ГОСТ 11371-78 4,3:1
- Совмещение:172 [Mate]: Винт 2 ГОСТ 17475-80 M4 x 14:2 ↔ Шайба  ГОСТ 11371-78 4,3:2
- Совмещение:173 [Mate]: BodyCupDiassembled:1 ↔ Шайба  ГОСТ 11371-78 4,3:2
- Совмещение:174 [Mate]: Винт 2 ГОСТ 17475-80 M4 x 14:4 ↔ Шайба  ГОСТ 11371-78 4,3:3
- Совмещение:175 [Mate]: BodyCupDiassembledMirroredMirrored:2 ↔ Шайба  ГОСТ 11371-78 4,3:3
- Совмещение:176 [Mate]: Винт 2 ГОСТ 17475-80 M4 x 14:3 ↔ Шайба  ГОСТ 11371-78 4,3:4
- Совмещение:177 [Mate]: BodyCupDiassembledMirroredMirrored:2 ↔ Шайба  ГОСТ 11371-78 4,3:4
- Совмещение:178 [Mate]: Винт 2 ГОСТ 17475-80 M4 x 14:5 ↔ Шайба  ГОСТ 11371-78 4,3:5
- Совмещение:179 [Mate]: BodyCupDiassembled:2 ↔ Шайба  ГОСТ 11371-78 4,3:5
- Совмещение:180 [Mate]: Винт 2 ГОСТ 17475-80 M4 x 14:6 ↔ Шайба  ГОСТ 11371-78 4,3:6
- Совмещение:181 [Mate]: BodyCupDiassembled:2 ↔ Шайба  ГОСТ 11371-78 4,3:6
- Совмещение:182 [Mate]: Винт 2 ГОСТ 17475-80 M4 x 14:7 ↔ Шайба  ГОСТ 11371-78 4,3:7
- Совмещение:183 [Mate]: BodyCupDiassembledMirroredMirrored:1 ↔ Шайба  ГОСТ 11371-78 4,3:7
- Совмещение:184 [Mate]: Винт 2 ГОСТ 17475-80 M4 x 14:8 ↔ Шайба  ГОСТ 11371-78 4,3:8
- Совмещение:185 [Mate]: BodyCupDiassembledMirroredMirrored:1 ↔ Шайба  ГОСТ 11371-78 4,3:8
- Совмещение:186 [Mate]: Винт 2 ГОСТ 17475-80 M4 x 14:7 ↔ DIN 934 - заменено на DIN EN 24032/28673/28674 M4:1
- Совмещение:187 [Mate]: Шайба  ГОСТ 11371-78 4,3:7 ↔ DIN 934 - заменено на DIN EN 24032/28673/28674 M4:1
- Совмещение:188 [Mate]: Винт 2 ГОСТ 17475-80 M4 x 14:8 ↔ DIN 934 - заменено на DIN EN 24032/28673/28674 M4:2
- Совмещение:189 [Mate]: Шайба  ГОСТ 11371-78 4,3:8 ↔ DIN 934 - заменено на DIN EN 24032/28673/28674 M4:2
- Совмещение:190 [Mate]: Винт 2 ГОСТ 17475-80 M4 x 14:6 ↔ DIN 934 - заменено на DIN EN 24032/28673/28674 M4:3
- Совмещение:191 [Mate]: Шайба  ГОСТ 11371-78 4,3:6 ↔ DIN 934 - заменено на DIN EN 24032/28673/28674 M4:3
- Совмещение:192 [Mate]: Винт 2 ГОСТ 17475-80 M4 x 14:5 ↔ DIN 934 - заменено на DIN EN 24032/28673/28674 M4:4
- Совмещение:193 [Mate]: Шайба  ГОСТ 11371-78 4,3:5 ↔ DIN 934 - заменено на DIN EN 24032/28673/28674 M4:4
- Совмещение:194 [Mate]: Винт 2 ГОСТ 17475-80 M4 x 14:2 ↔ DIN 934 - заменено на DIN EN 24032/28673/28674 M4:5
- Совмещение:195 [Mate]: Шайба  ГОСТ 11371-78 4,3:2 ↔ DIN 934 - заменено на DIN EN 24032/28673/28674 M4:5
- Совмещение:196 [Mate]: Винт 2 ГОСТ 17475-80 M4 x 14:1 ↔ DIN 934 - заменено на DIN EN 24032/28673/28674 M4:6
- Совмещение:197 [Mate]: Шайба  ГОСТ 11371-78 4,3:1 ↔ DIN 934 - заменено на DIN EN 24032/28673/28674 M4:6
- Совмещение:198 [Mate]: Винт 2 ГОСТ 17475-80 M4 x 14:4 ↔ DIN 934 - заменено на DIN EN 24032/28673/28674 M4:7
- Совмещение:199 [Mate]: Шайба  ГОСТ 11371-78 4,3:3 ↔ DIN 934 - заменено на DIN EN 24032/28673/28674 M4:7
- Совмещение:200 [Mate]: Винт 2 ГОСТ 17475-80 M4 x 14:3 ↔ DIN 934 - заменено на DIN EN 24032/28673/28674 M4:8
- Совмещение:201 [Mate]: Шайба  ГОСТ 11371-78 4,3:4 ↔ DIN 934 - заменено на DIN EN 24032/28673/28674 M4:8
## Named parameters: sa_0 = 452, sa_1 = 981, sa_2 = 1960
note: some values were not read from the file. Shown as the stored number, unit unknown: "sa_0", "sa_1", "sa_2".
